# Autodesk Inventor assembly: Assembly1
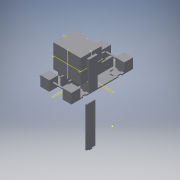
[picture p0: Inventor's stored thumbnail of the model, 180x180]
Saved by Autodesk Inventor 2018 (Build 220112000, 112)
## iProperties
Created: 2018-05-14
Part Number: Assembly1
Document SubType Name: Assembly
Designer: Administrator
Author: Administrator
## Documents named in this file (20)
- C:\Users\lenovo\Desktop\New folder\Assembly1.iam
- C:\Users\lenovo\Desktop\New folder\Part1.ipt
- C:\Users\lenovo\Desktop\New folder\Part2.ipt
- C:\Users\lenovo\Desktop\New folder\Part3.ipt
- C:\Users\lenovo\Desktop\New folder\Part4.ipt
- C:\Users\lenovo\Desktop\New folder\Part5.ipt
- C:\Users\lenovo\Desktop\New folder\Part6.ipt
- C:\Users\lenovo\Desktop\New folder\Part7.ipt
- C:\Users\lenovo\Desktop\New folder\Part8.ipt
- C:\Users\lenovo\Desktop\New folder\Part9.ipt
- C:\Users\lenovo\Desktop\New folder\Part10.ipt
- C:\Users\lenovo\Desktop\New folder\Part11.ipt
- C:\Users\lenovo\Desktop\New folder\Part12.ipt
- C:\Users\lenovo\Desktop\New folder\Part13.ipt
- C:\Users\lenovo\Desktop\New folder\Part14.ipt
- C:\Users\lenovo\Desktop\New folder\Part15.ipt
- C:\Users\lenovo\Desktop\New folder\Part16.ipt
- C:\Users\lenovo\Desktop\New folder\Part17.ipt
- C:\Users\lenovo\Desktop\New folder\Part18.ipt
- C:\Users\lenovo\Desktop\New folder\Part19.ipt
## Components (51 placed, 19 different names)
1. Part1:1 — Flush:49, Flush:50, Flush:51, Flush:52, Flush:53, Flush:54, Flush:55, Flush:56, Flush:57, Flush:58, Flush:59, Flush:60, Flush:61, Mate:1, Mate:2, Mate:3, Mate:4, Flush:62, Mate:5, Mate:6, Mate:7, Mate:8, Mate:12, Mate:13, Flush:93, Flush:96, Mate:16, Flush:112, Flush:113
2. Part2:1 — Flush:1, Flush:2, Flush:3, Flush:9, Flush:10, Flush:60, Insert:2
3. Part2:2 — Flush:4, Flush:5, Flush:6, Flush:7, Flush:8
4. Part3:1 — Flush:1, Flush:2, Flush:3, Flush:4, Flush:5, Flush:6, Flush:11, Flush:12
5. Part3:2 — Flush:7, Flush:8, Flush:9, Flush:56, Flush:57
6. Part4:1 — Flush:10, Flush:11, Flush:12
7. Part2:3
8. Part2:4 — Flush:59
9. Part3:3
10. Part3:4 — Flush:55, Flush:58
11. Part4:2
12. Part2:5 — Flush:54, Insert:1
13. Part2:6 — Flush:52
14. Part3:5 — Flush:53
15. Part3:6
16. Part4:3
17. Part2:7 — Flush:51
18. Part2:8 — Flush:50
19. Part3:7 — Flush:49
20. Part3:8
21. Part4:4
22. Part5:1 — Flush:61, Mate:1, Mate:2
23. Part5:2 — Mate:3, Mate:4, Flush:62
24. Part6:1 — Insert:2
25. Part6:2 — Insert:1
26. Part7:1 — Mate:5, Mate:6, Mate:7
27. Part8:1 — Flush:69, Flush:70, Flush:71, Flush:76, Flush:77, Mate:8
28. Part9:1 — Flush:66, Flush:67, Flush:68, Flush:72, Flush:75
29. Part10:1 — Flush:63, Flush:64, Flush:65, Flush:66, Flush:67, Flush:68, Flush:73, Flush:74
30. Part11:1 — Flush:63, Flush:64, Flush:65, Flush:69, Flush:70, Flush:71
31. Part12:1 — Flush:75, Flush:76, Flush:77, Mate:14, Mate:15, Flush:94
32. Part13:1 — Flush:72, Flush:73, Flush:74
33. Part14:1 — Flush:82, Flush:83, Mate:11
34. Part14:2 — Flush:78, Flush:79, Mate:9, Flush:80, Mate:10, Flush:81, Mate:15, Flush:99
35. Part15:1 — Flush:78, Flush:79, Mate:9, Mate:14
36. Part15:2 — Flush:80, Mate:10, Flush:81, Flush:82, Flush:83, Mate:11, Flush:94, Flush:98
37. Part4:5 — Flush:90, Flush:91, Flush:92
38. Part3:9 — Flush:84, Flush:85, Flush:86, Flush:87, Flush:88, Flush:89, Flush:92
39. Part3:10 — Flush:84, Flush:85, Flush:86, Flush:93, Flush:95
40. Part3:11 — Flush:87, Flush:88, Flush:89, Flush:90, Flush:91, Mate:12, Mate:13, Flush:97
41. Part16:1 — Flush:95, Flush:96, Flush:97, Flush:98, Flush:99
42. Part4:6
43. Part3:12
44. Part3:13 — Flush:111, Mate:16
45. Part3:14
46. Part16:2 — Flush:111, Flush:112, Flush:113, Flush:119, Flush:120, Flush:122
47. Part17:1 — Flush:114, Flush:115, Mate:17, Mate:19, Flush:121
48. Part18:1 — Flush:114, Flush:115, Mate:17, Flush:118
49. Part17:2 — Flush:118, Flush:122
50. Part18:2 — Mate:19, Flush:119, Flush:120, Flush:121
51. Part19:1
## Relationships (143: Flush 122, Mate 19, Insert 2)
- Flush:1: Part2:1 ↔ Part3:1
- Flush:2: Part2:1 ↔ Part3:1
- Flush:3: Part2:1 ↔ Part3:1
- Flush:4: Part2:2 ↔ Part3:1
- Flush:5: Part2:2 ↔ Part3:1
- Flush:6: Part2:2 ↔ Part3:1
- Flush:7: Part2:2 ↔ Part3:2
- Flush:8: Part2:2 ↔ Part3:2
- Flush:9: Part2:1 ↔ Part3:2
- Flush:10: Part2:1 ↔ Part4:1
- Flush:11: Part3:1 ↔ Part4:1
- Flush:12: Part3:1 ↔ Part4:1
- [Flush]: Part2:3 ↔ Part3:3
- [Flush]: Part2:3 ↔ Part3:3
- [Flush]: Part2:3 ↔ Part3:3
- [Flush]: Part2:4 ↔ Part3:3
- [Flush]: Part2:4 ↔ Part3:3
- [Flush]: Part2:4 ↔ Part3:3
- [Flush]: Part2:4 ↔ Part3:4
- [Flush]: Part2:4 ↔ Part3:4
- [Flush]: Part2:3 ↔ Part3:4
- [Flush]: Part2:3 ↔ Part4:2
- [Flush]: Part3:3 ↔ Part4:2
- [Flush]: Part3:3 ↔ Part4:2
- [Flush]: Part2:5 ↔ Part3:5
- [Flush]: Part2:5 ↔ Part3:5
- [Flush]: Part2:5 ↔ Part3:5
- [Flush]: Part2:6 ↔ Part3:5
- [Flush]: Part2:6 ↔ Part3:5
- [Flush]: Part2:6 ↔ Part3:5
- [Flush]: Part2:6 ↔ Part3:6
- [Flush]: Part2:6 ↔ Part3:6
- [Flush]: Part2:5 ↔ Part3:6
- [Flush]: Part2:5 ↔ Part4:3
- [Flush]: Part3:5 ↔ Part4:3
- [Flush]: Part3:5 ↔ Part4:3
- [Flush]: Part2:7 ↔ Part3:7
- [Flush]: Part2:7 ↔ Part3:7
- [Flush]: Part2:7 ↔ Part3:7
- [Flush]: Part2:8 ↔ Part3:7
- [Flush]: Part2:8 ↔ Part3:7
- [Flush]: Part2:8 ↔ Part3:7
- [Flush]: Part2:8 ↔ Part3:8
- [Flush]: Part2:8 ↔ Part3:8
- [Flush]: Part2:7 ↔ Part3:8
- [Flush]: Part2:7 ↔ Part4:4
- [Flush]: Part3:7 ↔ Part4:4
- [Flush]: Part3:7 ↔ Part4:4
- Flush:49: Part1:1 ↔ Part3:7
- Flush:50: Part1:1 ↔ Part2:8
- Flush:51: Part1:1 ↔ Part2:7
- Flush:52: Part1:1 ↔ Part2:6
- Flush:53: Part1:1 ↔ Part3:5
- Flush:54: Part1:1 ↔ Part2:5
- Flush:55: Part1:1 ↔ Part3:4
- Flush:56: Part1:1 ↔ Part3:2
- Flush:57: Part1:1 ↔ Part3:2
- Flush:58: Part1:1 ↔ Part3:4
- Flush:59: Part1:1 ↔ Part2:4
- Flush:60: Part1:1 ↔ Part2:1
- Flush:61: Part1:1 ↔ Part5:1
- Mate:1: Part1:1 ↔ Part5:1
- Mate:2: Part1:1 ↔ Part5:1
- Mate:3: Part1:1 ↔ Part5:2
- Mate:4: Part1:1 ↔ Part5:2
- Flush:62: Part1:1 ↔ Part5:2
- Insert:1: Part2:5 ↔ Part6:2
- Insert:2: Part2:1 ↔ Part6:1
- Mate:5: Part1:1 ↔ Part7:1
- Mate:6: Part1:1 ↔ Part7:1
- Mate:7: Part1:1 ↔ Part7:1
- Flush:63: Part10:1 ↔ Part11:1
- Flush:64: Part10:1 ↔ Part11:1
- Flush:65: Part10:1 ↔ Part11:1
- Flush:66: Part9:1 ↔ Part10:1
- Flush:67: Part9:1 ↔ Part10:1
- Flush:68: Part9:1 ↔ Part10:1
- Flush:69: Part8:1 ↔ Part11:1
- Flush:70: Part8:1 ↔ Part11:1
- Flush:71: Part8:1 ↔ Part11:1
- Flush:72: Part9:1 ↔ Part13:1
- Flush:73: Part10:1 ↔ Part13:1
- Flush:74: Part10:1 ↔ Part13:1
- Flush:75: Part9:1 ↔ Part12:1
- Flush:76: Part8:1 ↔ Part12:1
- Flush:77: Part8:1 ↔ Part12:1
- Mate:8 (25.4 mm): Part1:1 ↔ Part8:1
- Flush:78: Part14:2 ↔ Part15:1
- Flush:79: Part14:2 ↔ Part15:1
- Mate:9: Part14:2 ↔ Part15:1
- Flush:80: Part14:2 ↔ Part15:2
- Mate:10: Part14:2 ↔ Part15:2
- Flush:81: Part14:2 ↔ Part15:2
- Flush:82: Part14:1 ↔ Part15:2
- Flush:83: Part14:1 ↔ Part15:2
- Mate:11: Part14:1 ↔ Part15:2
- Flush:84: Part3:9 ↔ Part3:10
- Flush:85: Part3:9 ↔ Part3:10
- Flush:86: Part3:9 ↔ Part3:10
- Flush:87: Part3:9 ↔ Part3:11
- Flush:88: Part3:9 ↔ Part3:11
- Flush:89: Part3:9 ↔ Part3:11
- Flush:90: Part4:5 ↔ Part3:11
- Flush:91: Part4:5 ↔ Part3:11
- Flush:92: Part4:5 ↔ Part3:9
- Mate:12: Part1:1 ↔ Part3:11
- Mate:13: Part1:1 ↔ Part3:11
- Flush:93: Part1:1 ↔ Part3:10
- Mate:14: Part12:1 ↔ Part15:1
- Mate:15: Part12:1 ↔ Part14:2
- Flush:94: Part12:1 ↔ Part15:2
- Flush:95: Part3:10 ↔ Part16:1
- Flush:96: Part1:1 ↔ Part16:1
- Flush:97: Part3:11 ↔ Part16:1
- Flush:98: Part15:2 ↔ Part16:1
- Flush:99: Part14:2 ↔ Part16:1
- [Flush]: Part3:12 ↔ Part3:13
- [Flush]: Part3:12 ↔ Part3:13
- [Flush]: Part3:12 ↔ Part3:13
- [Flush]: Part3:12 ↔ Part3:14
- [Flush]: Part3:12 ↔ Part3:14
- [Flush]: Part3:12 ↔ Part3:14
- [Flush]: Part4:6 ↔ Part3:14
- [Flush]: Part4:6 ↔ Part3:14
- [Flush]: Part4:6 ↔ Part3:12
- [Flush]: Part3:13 ↔ Part16:2
- [Flush]: Part3:14 ↔ Part16:2
- Flush:111: Part3:13 ↔ Part16:2
- Mate:16: Part1:1 ↔ Part3:13
- Flush:112: Part1:1 ↔ Part16:2
- Flush:113: Part1:1 ↔ Part16:2
- Flush:114: Part17:1 ↔ Part18:1
- Flush:115: Part17:1 ↔ Part18:1
- Mate:17: Part17:1 ↔ Part18:1
- [Flush]: Part17:2 ↔ Part18:2
- [Flush]: Part17:2 ↔ Part18:2
- [Mate]: Part17:2 ↔ Part18:2
- Mate:19: Part17:1 ↔ Part18:2
- Flush:118: Part18:1 ↔ Part17:2
- Flush:119: Part16:2 ↔ Part18:2
- Flush:120: Part16:2 ↔ Part18:2
- Flush:121: Part17:1 ↔ Part18:2
- Flush:122: Part16:2 ↔ Part17:2
## Named parameters: d12_d1 = 0 mm, d13_d2 = 0 mm, d14_d3 = 0 mm, d15_d4 = 0 mm, d16_d5 = 0 mm, d17_d6 = 0 mm, d18_d7 = 0 mm, d19_d8 = 0 mm, d20_d9 = 0 mm, d21_d10 = 0 mm, d22_d11 = 0 mm, d23_d0 = 0 mm, d24_d1 = 0 mm, d25_d2 = 0 mm, d26_d3 = 0 mm, d27_d4 = 0 mm, d28_d5 = 0 mm, d29_d6 = 0 mm, d30_d7 = 0 mm, d31_d8 = 0 mm, d32_d9 = 0 mm, d33_d10 = 0 mm, d34_d11 = 0 mm, d35_d0 = 0 mm, d36_d1 = 0 mm, d37_d2 = 0 mm, d38_d3 = 0 mm, d39_d4 = 0 mm, d40_d5 = 0 mm, d41_d6 = 0 mm, d42_d7 = 0 mm, d43_d8 = 0 mm, d44_d9 = 0 mm, d45_d10 = 0 mm, d46_d11 = 0 mm, d47_d0 = 0 mm, d119_d99 = 0 mm, d120_d100 = 0 mm, d121_d101 = 0 mm, d122_d102 = 0 mm, d123_d103 = 0 mm, d124_d104 = 0 mm, d125_d105 = 0 mm, d126_d106 = 0 mm, d127_d107 = 0 mm, d128_d114 = 0 mm, d129_d116 = 0 mm, d137_d134 = 0 mm, d138_d135 = 0 mm, d139_d136 = 0 mm
